# Autodesk Inventor assembly: tip_ass_t1
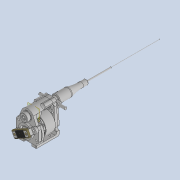
[picture p0: Inventor's stored thumbnail of the model, 180x180]
Saved by Autodesk Inventor 2020 (Build 240168000, 168)
## iProperties
Created: 2021-07-15
Part Number: tip_ass_t1
Document SubType Name: Assembly
Designer: Shuang Peng
Author: Shuang Peng
## Documents named in this file (14)
- D:\projects-3\torque fb tip\hardware\tip_ass_t1.iam
- D:\projects-3\torque fb tip\hardware\motor_1608.iam
- D:\projects-3\torque fb tip\hardware\pin_conn_1.ipt
- D:\projects-3\torque fb tip\hardware\bearing_3_6_2.ipt
- D:\projects-3\torque fb tip\hardware\pin_3_30.ipt
- D:\projects-3\torque fb tip\hardware\pin_fricition_ring_1.ipt
- D:\projects-3\torque fb tip\hardware\pin_conn_2.ipt
- D:\projects-3\torque fb tip\hardware\eletronic\as5600\as5600_tiny_3v3 v1\as5600_tiny_3v3.iam
- D:\projects-3\torque fb tip\hardware\ma_6.1_3_3.ipt
- D:\projects-3\torque fb tip\hardware\encoder_holder_1.ipt
- D:\projects-3\torque fb tip\hardware\ext_conn_1.ipt
- D:\projects-3\torque fb tip\hardware\needle_conn_1.ipt
- D:\projects-3\torque fb tip\hardware\neddle.ipt
- D:\projects-3\torque fb tip\hardware\Pin_2_8.ipt
## Components (18 placed, 13 different names)
1. motor_1608:1 [sub-assembly] — Flush:1, Insert:1, Insert:2, Insert:11
2. pin_conn_1:1 — Flush:1, Insert:1, Insert:2, Insert:9, Insert:10, Flush:3, Insert:13, Insert:14, Insert:21
3. bearing_3_6_2:1 — Insert:4, Insert:5, Insert:21
4. pin_3_30:1 — Insert:4, Insert:15
5. pin_fricition_ring_1:1 — Insert:6
6. pin_fricition_ring_1:2 — Insert:5, Insert:6
7. bearing_3_6_2:2 — Insert:8
8. bearing_3_6_2:3 — Insert:8, Flush:2, Insert:20
9. pin_conn_2:1 — Flush:2, Insert:9, Insert:10, Flush:4, Insert:16, Insert:17
10. as5600_tiny_3v3:1 [sub-assembly] — Angle:1
11. ma_6.1_3_3:1 — Insert:11
12. encoder_holder_1:1 — Flush:3, Angle:1, Insert:13, Insert:14
13. ma_6.1_3_3:2 — Insert:15
14. ext_conn_1:1 — Flush:4, Insert:16, Insert:17, Insert:18, Insert:20, Insert:22, Insert:23
15. needle_conn_1:1 — Insert:18, Insert:24
16. neddle:1 — Insert:24
17. Pin_2_8:1 — Insert:22
18. Pin_2_8:2 — Insert:23
## Relationships (25: Insert 20, Flush 4, Angle 1)
- Flush:1: motor_1608:1 ↔ pin_conn_1:1
- Insert:1: motor_1608:1 ↔ pin_conn_1:1
- Insert:2: motor_1608:1 ↔ pin_conn_1:1
- Insert:4 (-3 mm): bearing_3_6_2:1 ↔ pin_3_30:1
- Insert:5 (-6 mm): bearing_3_6_2:1 ↔ pin_fricition_ring_1:2
- Insert:6 (-3.5 mm): pin_fricition_ring_1:1 ↔ pin_fricition_ring_1:2
- Insert:8 (10 mm): bearing_3_6_2:2 ↔ bearing_3_6_2:3
- Flush:2: bearing_3_6_2:3 ↔ pin_conn_2:1
- Insert:9: pin_conn_1:1 ↔ pin_conn_2:1
- Insert:10: pin_conn_1:1 ↔ pin_conn_2:1
- Insert:11: motor_1608:1 ↔ ma_6.1_3_3:1
- Flush:3: pin_conn_1:1 ↔ encoder_holder_1:1
- Angle:1 (0 deg): as5600_tiny_3v3:1 ↔ encoder_holder_1:1
- Insert:13: pin_conn_1:1 ↔ encoder_holder_1:1
- Insert:14: pin_conn_1:1 ↔ encoder_holder_1:1
- Insert:15 (-0.5 mm): pin_3_30:1 ↔ ma_6.1_3_3:2
- Flush:4: pin_conn_2:1 ↔ ext_conn_1:1
- Insert:16: pin_conn_2:1 ↔ ext_conn_1:1
- Insert:17: pin_conn_2:1 ↔ ext_conn_1:1
- Insert:18 (0.5 mm): ext_conn_1:1 ↔ needle_conn_1:1
- Insert:20: bearing_3_6_2:3 ↔ ext_conn_1:1
- Insert:21: pin_conn_1:1 ↔ bearing_3_6_2:1
- Insert:22 (-3 mm): ext_conn_1:1 ↔ Pin_2_8:1
- Insert:23 (-3 mm): ext_conn_1:1 ↔ Pin_2_8:2
- Insert:24 (-20 mm): needle_conn_1:1 ↔ neddle:1
